# Autodesk Inventor assembly: Assembly1
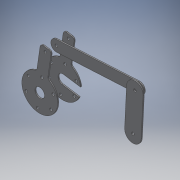
[picture p0: Inventor's stored thumbnail of the model, 180x180]
Saved by Autodesk Inventor 2016 (Build 200138000, 138)
## iProperties
Created: 2015-07-20
Part Number: Assembly1
Document SubType Name: Assembly
Designer: chdsbd
Author: chdsbd
## Documents named in this file (5)
- C:\Users\chdsbd\Dropbox\chris\projects\rfid_lock\models\clamp\clamp_assembly.iam
- C:\Users\chdsbd\Dropbox\chris\projects\rfid_lock\models\clamp\door_clamp.ipt
- C:\Users\chdsbd\Dropbox\chris\projects\rfid_lock\models\clamp\door_clamp_back.ipt
- C:\Users\chdsbd\Dropbox\chris\projects\rfid_lock\models\clamp\link.ipt
- C:\Users\chdsbd\Dropbox\chris\projects\rfid_lock\models\clamp\servo_arm.ipt
## Components (4 placed, 4 different names)
1. door_clamp:1 — Mate:1, Mate:3, Mate:5
2. door_clamp_back:1 — Mate:1, Mate:3, Mate:4, Mate:5, Mate:6
3. link:1 — Mate:4, Mate:6, Mate:7, Mate:8
4. servo_arm:1 — Mate:7, Mate:8
## Relationships (7: Mate 7)
- Mate:1: door_clamp:1 ↔ door_clamp_back:1
- Mate:3: door_clamp:1 ↔ door_clamp_back:1
- Mate:4: door_clamp_back:1 ↔ link:1
- Mate:5 (50.8 mm): door_clamp:1 ↔ door_clamp_back:1
- Mate:6 (25.4 mm): door_clamp_back:1 ↔ link:1
- Mate:7: link:1 ↔ servo_arm:1
- Mate:8 (6.35 mm): link:1 ↔ servo_arm:1
